# Autodesk Inventor assembly: Montagem
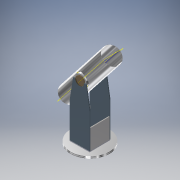
[picture p0: Inventor's stored thumbnail of the model, 180x180]
Saved by Autodesk Inventor 2016 (Build 200138000, 138)
## iProperties
Created: 2017-04-03
Part Number: Montagem
Document SubType Name: Assembly
Designer: Marcelo
Author: Marcelo
## Documents named in this file (8)
- D:\Users\Marcelo\Documents\GitHub\telescopiocaseiro\Hardware\PT-001\Montagem.iam
- D:\Users\Marcelo\Documents\GitHub\telescopiocaseiro\Hardware\PT-001\DiscoAzimute.ipt
- D:\Users\Marcelo\Documents\GitHub\telescopiocaseiro\Hardware\PT-001\Afastador.ipt
- D:\Users\Marcelo\Documents\GitHub\telescopiocaseiro\Hardware\PT-001\Suporte.ipt
- D:\Users\Marcelo\Documents\GitHub\telescopiocaseiro\Hardware\PT-001\Base.ipt
- D:\Users\Marcelo\Documents\GitHub\telescopiocaseiro\Hardware\PT-001\3rdParty\inafag_51112_wq8jww51abp3ix7r1ro4qx7x.iam
- D:\Users\Marcelo\Documents\GitHub\telescopiocaseiro\Hardware\PT-001\DiscoAzimuteBase.ipt
- D:\Users\Marcelo\Documents\GitHub\telescopiocaseiro\Hardware\PT-001\Montagem2.iam
## Components (9 placed, 7 different names)
1. DiscoAzimute:1 — Mate:9, Mate:10, Mate:11, Mate:12
2. Suporte:1 — Mate:4, Flush:7, Flush:8, Flush:10, Flush:11, Flush:12, Mate:7, Mate:16
3. Suporte:2 — Flush:5, Mate:5, Flush:6, Flush:9, Mate:6, Mate:15
4. Afastador:2 — Mate:4, Flush:5, Mate:5, Flush:6, Flush:7, Flush:8, Flush:9
5. Afastador:3 — Mate:6, Flush:10, Flush:11, Flush:13
6. Base:1 — Flush:12, Flush:13, Mate:7, Mate:9, Mate:10
7. inafag_51112_wq8jww51abp3ix7r1ro4qx7x:1 [sub-assembly] — Mate:11, Mate:12, Mate:13, Mate:14
8. DiscoAzimuteBase:1 — Mate:13, Mate:14
9. Montagem2:1 [sub-assembly] — Mate:15, Mate:16
## Relationships (21: Mate 12, Flush 9)
- Mate:4: Suporte:1 ↔ Afastador:2
- Flush:5: Suporte:2 ↔ Afastador:2
- Mate:5: Suporte:2 ↔ Afastador:2
- Flush:6: Suporte:2 ↔ Afastador:2
- Flush:7: Suporte:1 ↔ Afastador:2
- Flush:8: Suporte:1 ↔ Afastador:2
- Flush:9: Suporte:2 ↔ Afastador:2
- Mate:6: Suporte:2 ↔ Afastador:3
- Flush:10: Suporte:1 ↔ Afastador:3
- Flush:11: Suporte:1 ↔ Afastador:3
- Flush:12: Suporte:1 ↔ Base:1
- Flush:13: Afastador:3 ↔ Base:1
- Mate:7: Suporte:1 ↔ Base:1
- Mate:9: DiscoAzimute:1 ↔ Base:1
- Mate:10: DiscoAzimute:1 ↔ Base:1
- Mate:11: DiscoAzimute:1 ↔ inafag_51112_wq8jww51abp3ix7r1ro4qx7x:1
- Mate:12: DiscoAzimute:1 ↔ inafag_51112_wq8jww51abp3ix7r1ro4qx7x:1
- Mate:13: inafag_51112_wq8jww51abp3ix7r1ro4qx7x:1 ↔ DiscoAzimuteBase:1
- Mate:14: inafag_51112_wq8jww51abp3ix7r1ro4qx7x:1 ↔ DiscoAzimuteBase:1
- Mate:15: Suporte:2 ↔ Montagem2:1
- Mate:16 (5 mm): Suporte:1 ↔ Montagem2:1
